# Autodesk Inventor assembly: Tape Measure Bracket Assembly V5
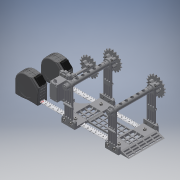
[picture p0: Inventor's stored thumbnail of the model, 180x180]
Saved by Autodesk Inventor 2019 (Build 230136000, 136)
## iProperties
Created: 2018-11-08
Part Number: Tape Measure Bracket Assembly V5
Document SubType Name: Assembly
Designer: Ashley
Author: Ashley
## Documents named in this file (32)
- C:\Users\Ashley\Desktop\repositories\design\inventor\2018-2019\Tape Measure Braket\Version Five\Tape Measure Bracket Assembly V5.1.iam
- C:\Users\Ashley\Desktop\repositories\design\inventor\2018-2019\Tape Measure Braket\Version Four\Bracket Bottom V4.ipt
- C:\Users\Ashley\Desktop\repositories\design\inventor\2018-2019\Tape Measure Braket\Tape Measure\Tape Measure Edited.iam
- C:\Users\Ashley\Desktop\repositories\design\inventor\2018-2019\Tape Measure Braket\Version Four\Side V4.ipt
- C:\Users\Ashley\Desktop\repositories\design\inventor\2018-2019\Tape Measure Braket\Version Two\Braket Top V2.ipt
- C:\Users\Ashley\Desktop\repositories\design\inventor\2018-2019\Tape Measure Braket\Version Five\Tape Measure Bracket Assembly V5\Design Accelerator\Bolted Connection2.iam
- C:\Users\Ashley\Desktop\repositories\design\inventor\2018-2019\Tape Measure Braket\Version Five\Tape Measure Bracket Assembly V5\Design Accelerator\Bolted Connection3.iam
- C:\Users\Ashley\Desktop\repositories\design\inventor\2018-2019\Tape Measure Braket\Version Five\Tape Measure Bracket Assembly V5\Design Accelerator\Bolted Connection4.iam
- C:\Users\Ashley\Desktop\repositories\design\inventor\2018-2019\Tape Measure Braket\Version Five\Tape Measure Bracket Assembly V5\Design Accelerator\Bolted Connection6.iam
- C:\Users\Ashley\Desktop\repositories\design\inventor\2018-2019\Tape Measure Braket\Version Five\Tape Measure Bracket Assembly V5\Design Accelerator\Bolted Connection7.iam
- C:\Users\Ashley\Desktop\repositories\design\inventor\2018-2019\Tape Measure Braket\Version Five\Tape Measure Bracket Assembly V5\Design Accelerator\Bolted Connection8.iam
- C:\Users\Ashley\Desktop\repositories\design\inventor\2018-2019\Tape Measure Braket\Version Five\Tape Measure Bracket Assembly V5\Design Accelerator\Bolted Connection9.iam
- C:\Users\Ashley\Desktop\repositories\design\inventor\2018-2019\Tape Measure Braket\Version Five\Tape Measure Bracket Assembly V5\Design Accelerator\Bolted Connection10.iam
- C:\Users\Ashley\Desktop\repositories\design\inventor\2018-2019\Tape Measure Braket\Version Five\Tape Measure Bracket Assembly V5\Design Accelerator\Bolted Connection11.iam
- C:\Users\Ashley\Desktop\repositories\design\inventor\2018-2019\Tape Measure Braket\Version Five\Tape Measure Bracket Assembly V5\Design Accelerator\Bolted Connection12.iam
- C:\Users\Ashley\Desktop\repositories\design\inventor\2018-2019\Tape Measure Braket\Version Five\Tape Measure Bracket Assembly V5\Design Accelerator\Bolted Connection13.iam
- C:\Users\Ashley\Desktop\repositories\design\inventor\Imported Components\goBilda\Bearing6mmID.ipt
- C:\Users\Ashley\Desktop\repositories\design\inventor\Imported Components\goBilda\DShaft30mm.ipt
- C:\Users\Ashley\Desktop\repositories\design\inventor\Imported Components\goBilda\Collar6mm\SetScrewCollar6mmboreassembly.iam
- C:\Users\Ashley\Desktop\repositories\design\inventor\2018-2019\Tape Measure Braket\Version Four\SpinnerV4.ipt
- C:\Users\Ashley\Desktop\repositories\design\inventor\Imported Components\goBilda\CampingHub\ClampingHub assembly.iam
- C:\Users\Ashley\Desktop\repositories\design\inventor\Imported Components\goBilda\8mmPlasticPitchSproket.ipt
- C:\Users\Ashley\Desktop\repositories\design\inventor\2018-2019\Tape Measure Braket\Version Five\Tape Measure Bracket Assembly V5\Design Accelerator\Bolted Connection14.iam
- C:\Users\Ashley\Desktop\repositories\design\inventor\2018-2019\Tape Measure Braket\Version Five\Tape Measure Bracket Assembly V5\Design Accelerator\Bolted Connection15.iam
- C:\Users\Ashley\Desktop\repositories\design\inventor\2018-2019\Tape Measure Braket\Version Five\Tape Measure Bracket Assembly V5\Design Accelerator\Bolted Connection16.iam
- C:\Users\Ashley\Desktop\repositories\design\inventor\2018-2019\Tape Measure Braket\Version Five\Tape Measure Bracket Assembly V5\Design Accelerator\Bolted Connection17.iam
- C:\Users\Ashley\Desktop\repositories\design\inventor\2018-2019\Tape Measure Braket\Version Five\Tape Measure Bracket Assembly V5\Design Accelerator\Bolted Connection18.iam
- C:\Users\Ashley\Desktop\repositories\design\inventor\Imported Components\goBilda\Servo and Frame.iam
- C:\Users\Ashley\Desktop\repositories\design\inventor\Imported Components\goBilda\Servo To Shaft\ServoToShaftCoupler.iam
- C:\Users\Ashley\Desktop\repositories\design\inventor\2018-2019\Tape Measure Braket\Version Five\Tape Measure Bracket Assembly V5\Design Accelerator\Bolted Connection20.iam
- C:\Users\Ashley\Desktop\repositories\design\inventor\Imported Components\goBilda\DShaft50mm.ipt
- C:\Users\Ashley\Desktop\repositories\design\inventor\2018-2019\Tape Measure Braket\Version Five\Tape Measure Bracket Assembly V5\Design Accelerator\Bolted Connection5.iam
## Components (58 placed, 15 different names)
1. Bracket Bottom — Mate:4, Mate:5, Insert:1, Insert:2, Insert:3, Insert:4, Insert:5, Insert:6, Insert:29, Mate:51, Mate:52
2. Tape Measure Right [sub-assembly]
3. Tape Measure Left [sub-assembly]
4. Braket Top V2:1 — Mate:5, Mate:22, Mate:23
5. Braket Top V2:2 — Mate:4, Mate:20, Mate:21
6. Braket Top V2:3 — Mate:26, Mate:27
7. Braket Top V2:4 — Mate:24, Mate:25
8. Side V4:1 — Insert:6, Mate:16, Mate:17, Mate:18, Mate:19, Insert:9
9. Side V4:2 — Insert:1, Insert:2, Mate:6, Mate:7, Insert:7
10. Side V4:3 — Insert:3, Insert:4, Mate:8, Mate:9, Mate:10, Mate:11, Mate:28
11. Side V4:4 — Insert:5, Mate:12, Mate:13, Mate:14, Mate:15, Insert:8
12. Bolted Connection:1 [sub-assembly] — Mate:6, Mate:7
13. Bolted Connection:2 [sub-assembly] — Mate:8, Mate:9
14. Bolted Connection:3 [sub-assembly] — Mate:10, Mate:11
15. Bolted Connection:4 [sub-assembly] — Mate:12, Mate:13
16. Bolted Connection:5 [sub-assembly] — Mate:14, Mate:15
17. Bolted Connection:6 [sub-assembly] — Mate:16, Mate:17
18. Bolted Connection:7 [sub-assembly] — Mate:18, Mate:19
19. Bolted Connection:8 [sub-assembly] — Mate:20, Mate:21
20. Bolted Connection:9 [sub-assembly] — Mate:22, Mate:23
21. Bolted Connection:10 [sub-assembly] — Mate:24, Mate:25
22. Bolted Connection:11 [sub-assembly] — Mate:26, Mate:27
23. Bearing6mmID:1 — Mate:28, Insert:12
24. Bearing6mmID:2 — Insert:8, Insert:13
25. Bearing6mmID:3 — Insert:7, Insert:11, Insert:24
26. Bearing6mmID:4 — Insert:9, Insert:10
27. DShaft30mm:1 — Insert:12, Insert:16, Insert:19
28. DShaft30mm:2 — Insert:13, Insert:15, Insert:20
29. DShaft30mm:3 — Insert:10, Insert:21, Insert:22, Insert:28
30. DShaft30mm:4 — Insert:11, Insert:18, Insert:23
31. SetScrewCollar6mmboreassembly:4 [sub-assembly] — Insert:16
32. SetScrewCollar6mmboreassembly:5 [sub-assembly] — Insert:15
33. SetScrewCollar6mmboreassembly:6 [sub-assembly] — Insert:18
34. SetScrewCollar6mmboreassembly:7 [sub-assembly] — Insert:21
35. SetScrewCollar6mmboreassembly:8 [sub-assembly] — Insert:19
36. SetScrewCollar6mmboreassembly:9 [sub-assembly] — Insert:20
37. SpinnerV4:1 — Insert:22
38. SpinnerV4:2 — Insert:23
39. ClampingHub assembly:3 [sub-assembly] — Insert:24, Insert:26
40. 8mmPlasticPitchSproket:1 — Insert:26, Mate:37, Mate:38
41. ClampingHub assembly:4 [sub-assembly] — Insert:28
42. 8mmPlasticPitchSproket:2 — Mate:29, Mate:30, Mate:31, Mate:32, Mate:33, Mate:34, Mate:35, Mate:36
43. Bolted Connection:12 [sub-assembly] — Mate:29, Mate:30
44. Bolted Connection:13 [sub-assembly] — Mate:31, Mate:32
45. Bolted Connection:14 [sub-assembly] — Mate:33, Mate:34
46. Bolted Connection:15 [sub-assembly] — Mate:35, Mate:36
47. Bolted Connection:16 [sub-assembly] — Mate:37, Mate:38
48. Servo and Frame:2 [sub-assembly] — Insert:29, Insert:30
49. ServoToShaftCoupler:1 [sub-assembly] — Insert:30, Mate:41, Mate:42, Insert:31
50. Bolted Connection:18 [sub-assembly] — Mate:41, Mate:42
51. DShaft50mm:1 — Insert:31, Insert:33
52. ClampingHub assembly:5 [sub-assembly] — Insert:33
53. 8mmPlasticPitchSproket:3
54. Bolted Connection:19 [sub-assembly]
55. Bolted Connection:20 [sub-assembly]
56. Bolted Connection:21 [sub-assembly]
57. Bolted Connection:22 [sub-assembly]
58. Bolted Connection:23 [sub-assembly] — Mate:51, Mate:52
## Relationships (77: Mate 47, Insert 30)
- Mate:4: Bracket Bottom ↔ Braket Top V2:2
- Mate:5: Bracket Bottom ↔ Braket Top V2:1
- Insert:1: Bracket Bottom ↔ Side V4:2
- Insert:2: Bracket Bottom ↔ Side V4:2
- Insert:3: Bracket Bottom ↔ Side V4:3
- Insert:4: Bracket Bottom ↔ Side V4:3
- Mate:6: Side V4:2 ↔ Bolted Connection:1
- Mate:7: Side V4:2 ↔ Bolted Connection:1
- Mate:8: Side V4:3 ↔ Bolted Connection:2
- Mate:9: Side V4:3 ↔ Bolted Connection:2
- Mate:10: Side V4:3 ↔ Bolted Connection:3
- Mate:11: Side V4:3 ↔ Bolted Connection:3
- Insert:5: Bracket Bottom ↔ Side V4:4
- Mate:12: Side V4:4 ↔ Bolted Connection:4
- Mate:13: Side V4:4 ↔ Bolted Connection:4
- Mate:14: Side V4:4 ↔ Bolted Connection:5
- Mate:15: Side V4:4 ↔ Bolted Connection:5
- Insert:6: Bracket Bottom ↔ Side V4:1
- Mate:16: Side V4:1 ↔ Bolted Connection:6
- Mate:17: Side V4:1 ↔ Bolted Connection:6
- Mate:18: Side V4:1 ↔ Bolted Connection:7
- Mate:19: Side V4:1 ↔ Bolted Connection:7
- Mate:20: Braket Top V2:2 ↔ Bolted Connection:8
- Mate:21: Braket Top V2:2 ↔ Bolted Connection:8
- Mate:22: Braket Top V2:1 ↔ Bolted Connection:9
- Mate:23: Braket Top V2:1 ↔ Bolted Connection:9
- Mate:24: Braket Top V2:4 ↔ Bolted Connection:10
- Mate:25: Braket Top V2:4 ↔ Bolted Connection:10
- Mate:26: Braket Top V2:3 ↔ Bolted Connection:11
- Mate:27: Braket Top V2:3 ↔ Bolted Connection:11
- Insert:7 (-3.55 mm): Side V4:2 ↔ Bearing6mmID:3
- Mate:28: Side V4:3 ↔ Bearing6mmID:1
- Insert:8 (-3.5 mm): Side V4:4 ↔ Bearing6mmID:2
- Insert:9 (-3.5 mm): Side V4:1 ↔ Bearing6mmID:4
- Insert:10 (9 mm): Bearing6mmID:4 ↔ DShaft30mm:3
- Insert:11 (16 mm): Bearing6mmID:3 ↔ DShaft30mm:4
- Insert:12 (9 mm): Bearing6mmID:1 ↔ DShaft30mm:1
- Insert:13 (9 mm): Bearing6mmID:2 ↔ DShaft30mm:2
- Insert:15 (0.7 mm): DShaft30mm:2 ↔ SetScrewCollar6mmboreassembly:5
- Insert:16 (0.6 mm): DShaft30mm:1 ↔ SetScrewCollar6mmboreassembly:4
- Insert:18 (7.4 mm): DShaft30mm:4 ↔ SetScrewCollar6mmboreassembly:6
- Insert:19 (8 mm): DShaft30mm:1 ↔ SetScrewCollar6mmboreassembly:8
- Insert:20 (7.7 mm): DShaft30mm:2 ↔ SetScrewCollar6mmboreassembly:9
- Insert:21 (7.8 mm): DShaft30mm:3 ↔ SetScrewCollar6mmboreassembly:7
- Insert:22 (-73 mm): DShaft30mm:3 ↔ SpinnerV4:1
- Insert:23 (-73.4 mm): DShaft30mm:4 ↔ SpinnerV4:2
- Insert:24 (0.5 mm): Bearing6mmID:3 ↔ ClampingHub assembly:3
- Insert:26 (-1 mm): ClampingHub assembly:3 ↔ 8mmPlasticPitchSproket:1
- [Insert] (-1 mm): ClampingHub assembly:4 ↔ 8mmPlasticPitchSproket:2
- Insert:28 (-8.6 mm): DShaft30mm:3 ↔ ClampingHub assembly:4
- Mate:29: 8mmPlasticPitchSproket:2 ↔ Bolted Connection:12
- Mate:30: 8mmPlasticPitchSproket:2 ↔ Bolted Connection:12
- Mate:31: 8mmPlasticPitchSproket:2 ↔ Bolted Connection:13
- Mate:32: 8mmPlasticPitchSproket:2 ↔ Bolted Connection:13
- Mate:33: 8mmPlasticPitchSproket:2 ↔ Bolted Connection:14
- Mate:34: 8mmPlasticPitchSproket:2 ↔ Bolted Connection:14
- Mate:35: 8mmPlasticPitchSproket:2 ↔ Bolted Connection:15
- Mate:36: 8mmPlasticPitchSproket:2 ↔ Bolted Connection:15
- Mate:37: 8mmPlasticPitchSproket:1 ↔ Bolted Connection:16
- Mate:38: 8mmPlasticPitchSproket:1 ↔ Bolted Connection:16
- Insert:29: Bracket Bottom ↔ Servo and Frame:2
- Insert:30: Servo and Frame:2 ↔ ServoToShaftCoupler:1
- Mate:41: ServoToShaftCoupler:1 ↔ Bolted Connection:18
- Mate:42: ServoToShaftCoupler:1 ↔ Bolted Connection:18
- Insert:31 (-10 mm): ServoToShaftCoupler:1 ↔ DShaft50mm:1
- [Insert] (-1 mm): ClampingHub assembly:5 ↔ 8mmPlasticPitchSproket:3
- [Mate]: 8mmPlasticPitchSproket:3 ↔ Bolted Connection:19
- [Mate]: 8mmPlasticPitchSproket:3 ↔ Bolted Connection:19
- [Mate]: 8mmPlasticPitchSproket:3 ↔ Bolted Connection:20
- [Mate]: 8mmPlasticPitchSproket:3 ↔ Bolted Connection:20
- [Mate]: 8mmPlasticPitchSproket:3 ↔ Bolted Connection:21
- [Mate]: 8mmPlasticPitchSproket:3 ↔ Bolted Connection:21
- [Mate]: 8mmPlasticPitchSproket:3 ↔ Bolted Connection:22
- [Mate]: 8mmPlasticPitchSproket:3 ↔ Bolted Connection:22
- Insert:33 (0.1 mm): DShaft50mm:1 ↔ ClampingHub assembly:5
- Mate:51: Bracket Bottom ↔ Bolted Connection:23
- Mate:52: Bracket Bottom ↔ Bolted Connection:23
## Named parameters: d144_d143 = -1 mm, d163_d152 = 0 mm, d164_d153 = 0 mm, d165_d150 = 0 mm, d166_d151 = 0 mm, d167_d148 = 0 mm, d168_d149 = 0 mm, d169_d146 = 0 mm, d170_d147 = 0 mm, d172_d144_d143 = -1 mm
